# Autodesk Inventor assembly: 2017 Robot
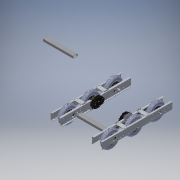
[picture p0: Inventor's stored thumbnail of the model, 180x180]
Saved by Autodesk Inventor 2016 (Build 200138000, 138)
## iProperties
Created: 2017-01-08
Part Number: 2017 Robot
Document SubType Name: Assembly
Designer: Dhruv
Author: Dhruv
## Documents named in this file (5)
- C:\Users\Dhruv\Desktop\MISC\FRC 2017\2017 Robot.iam
- C:\Users\Dhruv\Downloads\AM-14U3-PN8+Pneumatic+6WD.iam
- C:\Users\Dhruv\Desktop\MISC\FRC 2017\Tube.ipt
- C:\Users\Dhruv\Desktop\MISC\FRC 2017\90044A115_BLACK-OXIDE ALLOY STEEL SOCKET HEAD CAP SCREW.ipt
- C:\Users\Dhruv\Desktop\MISC\FRC 2017\94909A011_NYLON FLANGE NUTS.ipt
## Components (12 placed, 4 different names)
1. AM-14U3-PN8+Pneumatic+6WD:1 [sub-assembly] — Insert:1, Insert:7
2. AM-14U3-PN8+Pneumatic+6WD:2 [sub-assembly] — Insert:6, Insert:8, Insert:9
3. Tube:1
4. Tube:2 — Insert:1, Insert:2, Insert:3, Insert:4, Insert:5
5. 90044A115_BLACK-OXIDE ALLOY STEEL SOCKET HEAD CAP SCREW:1 — Insert:3
6. 90044A115_BLACK-OXIDE ALLOY STEEL SOCKET HEAD CAP SCREW:2 — Insert:2
7. 90044A115_BLACK-OXIDE ALLOY STEEL SOCKET HEAD CAP SCREW:3 — Insert:4
8. 90044A115_BLACK-OXIDE ALLOY STEEL SOCKET HEAD CAP SCREW:4 — Insert:5
9. 94909A011_NYLON FLANGE NUTS:1 — Insert:6
10. 94909A011_NYLON FLANGE NUTS:2 — Insert:8
11. 94909A011_NYLON FLANGE NUTS:3 — Insert:7
12. 94909A011_NYLON FLANGE NUTS:4 — Insert:9
## Relationships (9: Insert 9)
- Insert:1: AM-14U3-PN8+Pneumatic+6WD:1 ↔ Tube:2
- Insert:2: Tube:2 ↔ 90044A115_BLACK-OXIDE ALLOY STEEL SOCKET HEAD CAP SCREW:2
- Insert:3: Tube:2 ↔ 90044A115_BLACK-OXIDE ALLOY STEEL SOCKET HEAD CAP SCREW:1
- Insert:4: Tube:2 ↔ 90044A115_BLACK-OXIDE ALLOY STEEL SOCKET HEAD CAP SCREW:3
- Insert:5: Tube:2 ↔ 90044A115_BLACK-OXIDE ALLOY STEEL SOCKET HEAD CAP SCREW:4
- Insert:6: AM-14U3-PN8+Pneumatic+6WD:2 ↔ 94909A011_NYLON FLANGE NUTS:1
- Insert:7: AM-14U3-PN8+Pneumatic+6WD:1 ↔ 94909A011_NYLON FLANGE NUTS:3
- Insert:8: AM-14U3-PN8+Pneumatic+6WD:2 ↔ 94909A011_NYLON FLANGE NUTS:2
- Insert:9: AM-14U3-PN8+Pneumatic+6WD:2 ↔ 94909A011_NYLON FLANGE NUTS:4
